# Autodesk Inventor assembly: Scooter Assembly
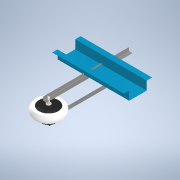
[picture p0: Inventor's stored thumbnail of the model, 180x180]
Saved by Autodesk Inventor 2021 (Build 250183000, 183)
## iProperties
Created: 2021-02-13
Part Number: Scooter Assembly
Document SubType Name: Assembly
Designer: bl17
Author: bl17
## Documents named in this file (5)
- P:\Personal Docs\Aubrey Scooter\Scooter Assembly.iam
- P:\Personal Docs\Aubrey Scooter\Cubby Sheet Metal.ipt
- P:\Personal Docs\Aubrey Scooter\Right Frame Iron.ipt
- P:\Personal Docs\Aubrey Scooter\Left Frame Iron.ipt
- \\prism.nas.gatech.edu\bl17\vlab\downloads\002. DC Brushed Wheels.ipt
## Components (4 placed, 4 different names)
1. Cubby Sheet Metal:1
2. Right Frame Iron:1 — Flush:1, Mate:1, Flush:2, Insert:1
3. Left Frame Iron:1 — Flush:1, Mate:1, Flush:2, Insert:2
4. 002. DC Brushed Wheels:1 — Insert:1, Insert:2
## Relationships (5: Flush 2, Insert 2, Mate 1)
- Flush:1: Right Frame Iron:1 ↔ Left Frame Iron:1
- Mate:1 (120 mm): Right Frame Iron:1 ↔ Left Frame Iron:1
- Flush:2: Right Frame Iron:1 ↔ Left Frame Iron:1
- Insert:1: Right Frame Iron:1 ↔ 002. DC Brushed Wheels:1
- Insert:2: Left Frame Iron:1 ↔ 002. DC Brushed Wheels:1
## Named parameters: axle_inset_fwd = 19.05 mm, axle_inset_up = 17.78 mm
